# Autodesk Inventor assembly: DriveChain2
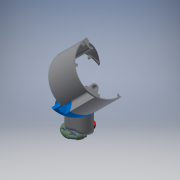
[picture p0: Inventor's stored thumbnail of the model, 180x180]
Saved by Autodesk Inventor 2019.1 (Build 231200000, 200)
## iProperties
Created: 2018-07-27
Part Number: DriveChain2
Material: Generisch
Document SubType Name: Assembly
Designer: JochenAlt
Author: JochenAlt
## Documents named in this file (10)
- D:\Projects\Ondine\CAD\DriveChain.iam
- D:\Projects\Ondine\CAD\BushOmniWheel.ipt
- D:\Projects\Ondine\CAD\Encoder\Avago Encoder.iam
- D:\Projects\Ondine\CAD\DriveChainEnclosure.ipt
- D:\Projects\Ondine\CAD\BeltDriveAxis.ipt
- D:\Projects\Ondine\CAD\BushBeltDriveTL.ipt
- D:\Projects\Ondine\CAD\Bearings\W 637_4 X-2Z.iam
- D:\Projects\Ondine\CAD\OmniWheel.iam
- D:\Projects\Ondine\CAD\Beltdrive\BeltGear.iam
- D:\Projects\Ondine\CAD\BeltDriveAxisSleeve.ipt
## Components (13 placed, 8 different names)
1. DriveChainEnclosure:1 — Passend:105, Passend:106, Passend:130, Passend:131, Passend:133, Passend:134, Passend:135, Passend:136
2. W 637_4 X-2Z:3 [sub-assembly] — Passend:130, Passend:131
3. W 637_4 X-2Z:2 [sub-assembly]
4. W 637_4 X-2Z:1 [sub-assembly] — Passend:105, Passend:106, Passend:119, Passend:140, Passend:149
5. BushOmniWheel:4 — Passend:119, Passend:128, Passend:140
6. BushOmniWheel:3 — Passend:80
7. BeltdriveAxis — Passend:80, Passend:132, Passend:133, Passend:136, Passend:137, Passend:138
8. Avago Encoder:1 [sub-assembly] — Winkel:1, Passend:142, Passend:143, Passend:144, Passend:145
9. BushOmniWheel:1 — Passend:147, Passend:148, Passend:149
10. OmniWheel:1 [sub-assembly] — Passend:141, Passend:146, Passend:148
11. W 637_4 X-2Z:4 [sub-assembly] — Passend:132, Passend:134, Passend:135
12. NewBeltGear:1 [sub-assembly] — Passend:128, Passend:137, Passend:139, Passend:141, Passend:142, Passend:143, Passend:144, Passend:145, Passend:146, Passend:147
13. BeltDriveAxisSleeve:1 — Passend:138, Passend:139
## Relationships (26: Mate 25, Angle 1)
- Passend:80 [Mate]: BushOmniWheel:3 ↔ BeltdriveAxis
- Winkel:1 [Angle] (90 deg): Avago Encoder:1
- Passend:105 [Mate]: DriveChainEnclosure:1 ↔ W 637_4 X-2Z:1
- Passend:106 [Mate]: DriveChainEnclosure:1 ↔ W 637_4 X-2Z:1
- Passend:119 [Mate]: W 637_4 X-2Z:1 ↔ BushOmniWheel:4
- Passend:128 [Mate]: BushOmniWheel:4 ↔ NewBeltGear:1
- Passend:130 [Mate]: DriveChainEnclosure:1 ↔ W 637_4 X-2Z:3
- Passend:131 [Mate]: DriveChainEnclosure:1 ↔ W 637_4 X-2Z:3
- Passend:132 [Mate]: BeltdriveAxis ↔ W 637_4 X-2Z:4
- Passend:133 [Mate]: DriveChainEnclosure:1 ↔ BeltdriveAxis
- Passend:134 [Mate]: DriveChainEnclosure:1 ↔ W 637_4 X-2Z:4
- Passend:135 [Mate]: DriveChainEnclosure:1 ↔ W 637_4 X-2Z:4
- Passend:136 [Mate]: DriveChainEnclosure:1 ↔ BeltdriveAxis
- Passend:137 [Mate]: BeltdriveAxis ↔ NewBeltGear:1
- Passend:138 [Mate]: BeltdriveAxis ↔ BeltDriveAxisSleeve:1
- Passend:139 [Mate]: NewBeltGear:1 ↔ BeltDriveAxisSleeve:1
- Passend:140 [Mate]: W 637_4 X-2Z:1 ↔ BushOmniWheel:4
- Passend:141 [Mate]: OmniWheel:1 ↔ NewBeltGear:1
- Passend:142 [Mate]: Avago Encoder:1 ↔ NewBeltGear:1
- Passend:143 [Mate]: Avago Encoder:1 ↔ NewBeltGear:1
- Passend:144 [Mate]: Avago Encoder:1 ↔ NewBeltGear:1
- Passend:145 [Mate]: Avago Encoder:1 ↔ NewBeltGear:1
- Passend:146 [Mate]: OmniWheel:1 ↔ NewBeltGear:1
- Passend:147 [Mate]: BushOmniWheel:1 ↔ NewBeltGear:1
- Passend:148 [Mate]: BushOmniWheel:1 ↔ OmniWheel:1
- Passend:149 [Mate]: W 637_4 X-2Z:1 ↔ BushOmniWheel:1
